# Autodesk Inventor assembly: mppcInterface
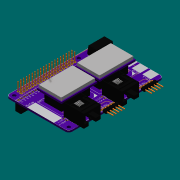
[picture p0: Inventor's stored thumbnail of the model, 180x180]
Saved by Autodesk Inventor 2016 SP1 (Build 200210100, 210)
## iProperties
Created: 2016-04-06
Part Number: mppcInterface
Document SubType Name: Assembly
Designer: sawai
Author: sawai
## Documents named in this file (8)
- C:\Users\sawai\OneDrive\projects\mppcInterface\cad\mppcInterface.iam
- C:\Users\sawai\OneDrive\projects\mppcInterface\cad\mppcInterfacePcb.ipt
- C:\Users\sawai\OneDrive\projects\mppcInterface\cad\connector\2.54Header\rightAngle\1x5Angle.iam
- C:\Users\sawai\OneDrive\projects\mppcInterface\cad\connector\8P8C.ipt
- C:\Users\sawai\OneDrive\projects\mppcInterface\cad\connector\2.54Header\piExtraTall\2x20ExtraTallHeader.iam
- C:\Users\sawai\OneDrive\projects\mppcInterface\cad\connector\2.54Header\female\1x6Female.iam
- C:\Users\sawai\OneDrive\projects\mppcInterface\cad\electronics\PDS1-M.ipt
- C:\Users\sawai\OneDrive\projects\mppcInterface\cad\dependency\mppcHighVoltage\cad\highVoltageMppc.iam
## Components (13 placed, 7 different names)
1. mppcInterfacePcb:1 — Mate:1, Angle:1, Mate:2, Mate:3, Angle:3, Mate:4, Angle:5, Mate:6, Mate:7, Mate:8, Angle:6
2. 1x5Angle:1 [sub-assembly] — Mate:1, Angle:1, Angle:2, Flush:2
3. 1x5Angle:2 [sub-assembly] — Angle:2, Mate:2, Flush:2
4. 8P8C:1 — Mate:3, Angle:3, Angle:4, Flush:1
5. 8P8C:2 — Angle:4, Mate:4, Flush:1
6. 2x20ExtraTallHeader:1 [sub-assembly] — Angle:5, Mate:7
7. 1x6Female:1 [sub-assembly] — Flush:3, Flush:8, Flush:15, Flush:16
8. 1x6Female:2 [sub-assembly] — Flush:3, Flush:4, Flush:7, Flush:8, Flush:11, Flush:12
9. 1x6Female:3 [sub-assembly] — Flush:4, Flush:5, Flush:6, Flush:7, Mate:10, Flush:13, Flush:14
10. 1x6Female:4 [sub-assembly] — Flush:5, Flush:6, Mate:6, Mate:9, Angle:7, Flush:9, Flush:10
11. PDS1-M:1 — Mate:8, Angle:6
12. highVoltageMppc:1 [sub-assembly] — Mate:9, Angle:7, Flush:9, Flush:10, Flush:11, Flush:12
13. highVoltageMppc:2 [sub-assembly] — Mate:10, Flush:13, Flush:14, Flush:15, Flush:16
## Relationships (32: Flush 16, Mate 9, Angle 7)
- Mate:1: mppcInterfacePcb:1 ↔ 1x5Angle:1
- Angle:1 (0 deg): mppcInterfacePcb:1 ↔ 1x5Angle:1
- Angle:2 (0 deg): 1x5Angle:1 ↔ 1x5Angle:2
- Mate:2: mppcInterfacePcb:1 ↔ 1x5Angle:2
- Mate:3: mppcInterfacePcb:1 ↔ 8P8C:1
- Angle:3 (0 deg): mppcInterfacePcb:1 ↔ 8P8C:1
- Angle:4 (0 deg): 8P8C:1 ↔ 8P8C:2
- Mate:4: mppcInterfacePcb:1 ↔ 8P8C:2
- Flush:1: 8P8C:1 ↔ 8P8C:2
- Flush:2: 1x5Angle:1 ↔ 1x5Angle:2
- Angle:5 (0 deg): mppcInterfacePcb:1 ↔ 2x20ExtraTallHeader:1
- Flush:3: 1x6Female:1 ↔ 1x6Female:2
- Flush:4: 1x6Female:2 ↔ 1x6Female:3
- Flush:5: 1x6Female:3 ↔ 1x6Female:4
- Flush:6: 1x6Female:3 ↔ 1x6Female:4
- Flush:7: 1x6Female:2 ↔ 1x6Female:3
- Flush:8: 1x6Female:1 ↔ 1x6Female:2
- Mate:6: mppcInterfacePcb:1 ↔ 1x6Female:4
- Mate:7: mppcInterfacePcb:1 ↔ 2x20ExtraTallHeader:1
- Mate:8: mppcInterfacePcb:1 ↔ PDS1-M:1
- Angle:6 (0 deg): mppcInterfacePcb:1 ↔ PDS1-M:1
- Mate:9: 1x6Female:4 ↔ highVoltageMppc:1
- Angle:7 (0 deg): 1x6Female:4 ↔ highVoltageMppc:1
- Flush:9: 1x6Female:4 ↔ highVoltageMppc:1
- Flush:10: 1x6Female:4 ↔ highVoltageMppc:1
- Flush:11: 1x6Female:2 ↔ highVoltageMppc:1
- Flush:12: 1x6Female:2 ↔ highVoltageMppc:1
- Mate:10: 1x6Female:3 ↔ highVoltageMppc:2
- Flush:13: 1x6Female:3 ↔ highVoltageMppc:2
- Flush:14: 1x6Female:3 ↔ highVoltageMppc:2
- Flush:15: 1x6Female:1 ↔ highVoltageMppc:2
- Flush:16: 1x6Female:1 ↔ highVoltageMppc:2
